# Autodesk Inventor assembly: Bat_claw_print
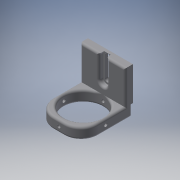
[picture p0: Inventor's stored thumbnail of the model, 180x180]
Saved by Autodesk Inventor 2019.3 (Build 233278000, 278)
## iProperties
Created: 2020-09-10
Part Number: Bat_claw_print
Material: Generisch
Document SubType Name: Assembly
Designer: Nicolas Frick
Author: Nicolas Frick
## Documents named in this file (2)
- C:\Users\Nicolas Frick\Sync\OneDrive\airhockeybot\mechanical_design\common_cad_parts\print_models\upper\Bat_claw_print.iam
- C:\Users\Nicolas Frick\Sync\OneDrive\airhockeybot\mechanical_design\inventor\Bat_claw.ipt
## Components (1 placed, 1 different names)
1. Bat_claw:1 — Passend:1, Passend:2, Fluchtend:1
## Relationships (3: Mate 2, Flush 1)
- Passend:1 [Mate]: Bat_claw:1
- Passend:2 [Mate]: Bat_claw:1
- Fluchtend:1 [Flush]: Bat_claw:1
